# Autodesk Inventor assembly: Assembly_Kolbentank
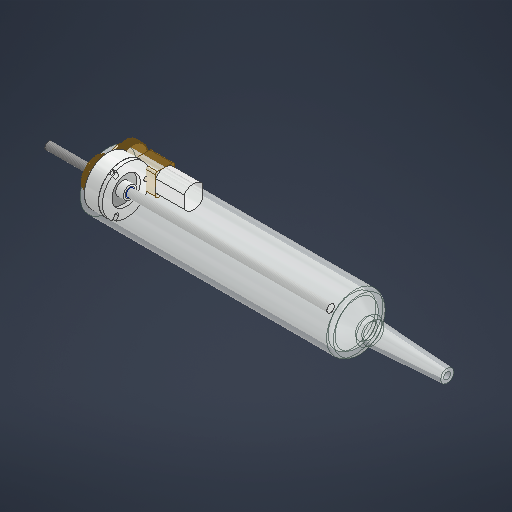
[picture p0: Inventor's stored thumbnail of the model, 512x512]
Saved by Autodesk Inventor 2026 (Build 300175000, 175)
## iProperties
Created: 2025-04-25
Part Number: Assembly_Kolbentank
Document SubType Name: Assembly
Designer: FAL
Author: FAL
## Documents named in this file (10)
- C:\Users\FAL\Desktop\git\U-BERT\CAD\Kolbentank\A_Kolbentank.iam
- C:\Users\FAL\Desktop\git\U-BERT\CAD\Kolbentank\P_Spritze_60ml.ipt
- C:\Users\FAL\Desktop\git\U-BERT\CAD\Kolbentank\P_Lagerschale.ipt
- C:\Users\FAL\Desktop\git\U-BERT\CAD\Kolbentank\P_Lager_19x6_5.ipt
- C:\Users\FAL\Desktop\git\U-BERT\CAD\Kolbentank\P_Lagerschale_Deckel.ipt
- C:\Users\FAL\Desktop\git\U-BERT\CAD\Kolbentank\P_Gewindestange_M4_150mm.ipt
- C:\Users\FAL\Desktop\git\U-BERT\CAD\Kolbentank\P_Gewindemotor_N20.ipt
- C:\Users\FAL\Desktop\git\U-BERT\CAD\Kolbentank\P_Gewindebuchse_M4_20.ipt
- C:\Users\FAL\Desktop\git\U-BERT\CAD\Kolbentank\P_Stellring_7x4_5.ipt
- C:\Users\FAL\Desktop\git\U-BERT\CAD\Kolbentank\P_Zahnrad.ipt
## Components (10 placed, 9 different names)
1. P_Spritze_60ml:1 — Fluchtend:2, Fluchtend:3, Fluchtend:4, Einfügen:1
2. P_Lagerschale:1 — Einfügen:1, Einfügen:2, Einfügen:3
3. P_Lager_19x6_5:1 — Einfügen:2, Zylindrisch:1, Einfügen:5, Passend:10, Passend:11
4. P_Lagerschale_Deckel:1 — Einfügen:3, Passend:6
5. P_Gewindestange_M4_150mm:1 — Zylindrisch:1
6. P_Gewindemotor_N20:1 — Passend:8
7. P_Gewindebuchse_M4_20:1 — Passend:7, Passend:9, Passend:10
8. P_Stellring_7x4_5:1 — Einfügen:5, Passend:7
9. P_Zahnrad:1 — Passend:8, Fluchtend:5
10. P_Zahnrad:2 — Passend:9, Passend:11, Fluchtend:5
## Relationships (15: Mate 6, Flush 4, Insert 4, CylindricalJoint 1)
- Fluchtend:2 [Flush]: P_Spritze_60ml:1
- Fluchtend:3 [Flush]: P_Spritze_60ml:1
- Fluchtend:4 [Flush]: P_Spritze_60ml:1
- Einfügen:1 [Insert]: P_Spritze_60ml:1 ↔ P_Lagerschale:1
- Einfügen:2 [Insert]: P_Lagerschale:1 ↔ P_Lager_19x6_5:1
- Einfügen:3 [Insert]: P_Lagerschale:1 ↔ P_Lagerschale_Deckel:1
- Passend:6 [Mate]: P_Lagerschale_Deckel:1
- Zylindrisch:1 [CylindricalJoint]: P_Lager_19x6_5:1 ↔ P_Gewindestange_M4_150mm:1
- Einfügen:5 [Insert]: P_Lager_19x6_5:1 ↔ P_Stellring_7x4_5:1
- Passend:7 [Mate]: P_Gewindebuchse_M4_20:1 ↔ P_Stellring_7x4_5:1
- Passend:8 [Mate]: P_Gewindemotor_N20:1 ↔ P_Zahnrad:1
- Passend:9 [Mate]: P_Gewindebuchse_M4_20:1 ↔ P_Zahnrad:2
- Passend:10 [Mate]: P_Lager_19x6_5:1 ↔ P_Gewindebuchse_M4_20:1
- Passend:11 [Mate]: P_Lager_19x6_5:1 ↔ P_Zahnrad:2
- Fluchtend:5 [Flush]: P_Zahnrad:1 ↔ P_Zahnrad:2
